# Autodesk Inventor assembly: Assembly1
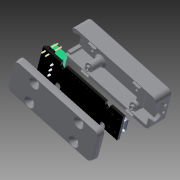
[picture p0: Inventor's stored thumbnail of the model, 180x180]
Saved by Autodesk Inventor 2014 SP2 (Build 180246200, 246)
## iProperties
Created: 2025-01-23
Part Number: Assembly1
Document SubType Name: Assembly
Designer: GauchoHP
Author: GauchoHP
## Documents named in this file (4)
- E:\Dati\Documenti_Emanuele\Linguaggi_di_Programmazione\ST MCU\baccable\canable\CANableAndLedsStripController\hardware\box\single fysect ucan\Assembly1.iam
- E:\Dati\Documenti_Emanuele\Linguaggi_di_Programmazione\ST MCU\baccable\canable\CANableAndLedsStripController\hardware\box\dual fysect ucan\dualBaccable-ucan_fysect.ipt
- E:\Dati\Documenti_Emanuele\Linguaggi_di_Programmazione\ST MCU\baccable\canable\CANableAndLedsStripController\hardware\box\dual fysect ucan\Imported Components\UCAN_ V1.0\UCAN_ V1.0.iam
- E:\Dati\Documenti_Emanuele\Linguaggi_di_Programmazione\ST MCU\baccable\canable\CANableAndLedsStripController\hardware\box\dual fysect ucan\singleBaccable-ucan_fysect_CAP.ipt
## Components (3 placed, 3 different names)
1. dualBaccable-ucan_fysect:1 — Mate:1, Mate:2, Mate:3
2. UCAN_ V1.0:1 [sub-assembly] — Mate:1, Mate:2, Mate:3, Mate:4, Mate:5, Mate:6
3. singleBaccable-ucan_fysect_CAP:1 — Mate:4, Mate:5, Mate:6
## Relationships (6: Mate 6)
- Mate:1: dualBaccable-ucan_fysect:1 ↔ UCAN_ V1.0:1
- Mate:2 (0.254 mm): dualBaccable-ucan_fysect:1 ↔ UCAN_ V1.0:1
- Mate:3 (17.5768 mm): dualBaccable-ucan_fysect:1 ↔ UCAN_ V1.0:1
- Mate:4: UCAN_ V1.0:1 ↔ singleBaccable-ucan_fysect_CAP:1
- Mate:5 (0.254 mm): UCAN_ V1.0:1 ↔ singleBaccable-ucan_fysect_CAP:1
- Mate:6 (15.0114 mm): UCAN_ V1.0:1 ↔ singleBaccable-ucan_fysect_CAP:1
